# Autodesk Inventor assembly: GP5-200
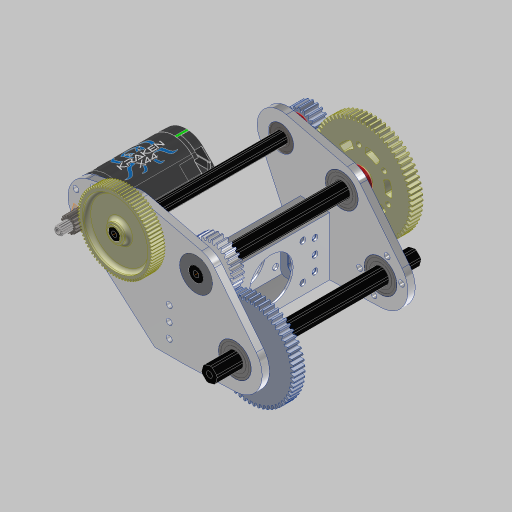
[picture p0: Inventor's stored thumbnail of the model, 512x512]
Saved by Autodesk Inventor 2023.5 (Build 275446000, 446)
## iProperties
Created: 2025-02-04
Part Number: GP5-200
Document SubType Name: Assembly
Designer: mavericks
Mass: 1428.35 g
Surface Area: 2144.98 cm^2
Volume: 477.65 cm^3
Density: 2.99036 g/cm^3
Author: mavericks
## Documents named in this file (21)
- C:\Users\slick\OneDrive\Desktop\2025-ReefScape---CAD\Gripper\GP5\GP5-200.iam
- C:\Users\slick\OneDrive\Desktop\2025-ReefScape---CAD\Gripper\GP5\GP5-001.ipt
- C:\Users\slick\OneDrive\Desktop\2025-ReefScape---CAD\Gripper\GP5\GP5-002.ipt
- C:\Users\slick\OneDrive\Desktop\2025-ReefScape---CAD\Gripper\GP5\GP5-004.ipt
- C:\Users\slick\OneDrive\Desktop\2025-ReefScape---CAD\COMMON PARTS\BEARINGS\13_75mm_1_2_ThunderHex_ID_x_1_125_OD_x_0_313_WD_Flanged_Bearing_217-4006_MIR.ipt
- C:\Users\slick\OneDrive\Desktop\2025-ReefScape---CAD\COMMON PARTS\MOTORS\WCP-0941 x44 Kracken.ipt
- C:\Users\slick\OneDrive\Desktop\2025-ReefScape---CAD\COMMON PARTS\GEARS\32 dp gear\WCP-1464.ipt
- C:\Users\slick\OneDrive\Desktop\2025-ReefScape---CAD\COMMON PARTS\GEARS\32 dp gear\80t_Aluminum_Spur_Gear_32_DP_3_8_Hex_Bore_217-5864.ipt
- C:\Users\slick\OneDrive\Desktop\2025-ReefScape---CAD\COMMON PARTS\GEARS\20dp .375 hex\20t_Aluminum_Spur_Gear_20_DP_3_8_Hex_Bore_217-2701.ipt
- C:\Users\slick\OneDrive\Desktop\2025-ReefScape---CAD\COMMON PARTS\GEARS\20dp .5 hex\66t_Aluminum_Spur_Gear_20_DP_1_2_Hex_Bore_VersaKeys_217-3223.ipt
- C:\Users\slick\OneDrive\Desktop\2025-ReefScape---CAD\COMMON PARTS\GEARS\20dp .5 hex\30t_Aluminum_Spur_Gear_20_DP_1_2_Hex_Bore_217-2705.ipt
- C:\Users\slick\OneDrive\Desktop\2025-ReefScape---CAD\COMMON PARTS\GEARS\20dp .5 hex\60t_Aluminum_Spur_Gear_20_DP_1_2_Hex_Bore_217-3574.ipt
- C:\Users\slick\OneDrive\Desktop\2025-ReefScape---CAD\Gripper\GP5\GP5-008.ipt
- C:\Users\slick\OneDrive\Desktop\2025-ReefScape---CAD\COMMON PARTS\BEARINGS\10_25mm_3_8_ThunderHex_ID_x_0_875_OD_x_0_280_WD_Flanged_Bearing_217-5829.ipt
- C:\Users\slick\OneDrive\Desktop\2025-ReefScape---CAD\Gripper\GP5\GP5-009.ipt
- C:\Users\slick\OneDrive\Desktop\2025-ReefScape---CAD\Gripper\GP5\GP5-010.ipt
- C:\Users\slick\OneDrive\Desktop\2025-ReefScape---CAD\Gripper\GP5\GP5-011.ipt
- C:\Users\slick\OneDrive\Desktop\2025-ReefScape---CAD\Gripper\GP5\GP5-020.ipt
- C:\Users\slick\OneDrive\Desktop\2025-ReefScape---CAD\Gripper\GP5\GP5-021.ipt
- C:\Users\slick\OneDrive\Desktop\2025-ReefScape---CAD\Gripper\GP5\GP5-022.ipt
- C:\Users\slick\OneDrive\Desktop\2025-ReefScape---CAD\COMMON PARTS\BEARINGS\0_500_ID_x_1_125_OD_x_0_313_WD_Flanged_Bearing_217-2731.ipt
## Components (26 placed, 20 different names)
1. GP5-001:1 — Flush:1, Flush:2, Flush:3, Flush:4, Flush:5, Mate:1
2. GP5-002:1 — Flush:2, Flush:3, Flush:4, Insert:3, Insert:4
3. GP5-002:2 — Flush:1, Flush:5, Mate:1, Insert:1, Insert:2
4. GP5-011:1 — Insert:3, Insert:4, Insert:5, Insert:6, Insert:13, Symmetry:1
5. GP5-004:2 — Insert:1, Insert:2, Insert:10, Mate:2, Mate:3, Insert:11, Insert:12, Insert:14, Symmetry:1
6. 0_500_ID_x_1_125_OD_x_0_313_WD_Flanged_Bearing_217-2731:1 — Insert:14, Flush:14, Mate:32, Mate:33
7. 13_75mm_1_2_ThunderHex_ID_x_1_125_OD_x_0_313_WD_Flanged_Bearing_217-4006_MIR:3 — Insert:10, Mate:12
8. 13_75mm_1_2_ThunderHex_ID_x_1_125_OD_x_0_313_WD_Flanged_Bearing_217-4006_MIR:5 — Insert:6, Mate:8, Mate:17, Mate:24
9. 13_75mm_1_2_ThunderHex_ID_x_1_125_OD_x_0_313_WD_Flanged_Bearing_217-4006_MIR:6 — Insert:5, Mate:18
10. WCP-0941 x44 Kracken:1 — Mate:2, Mate:3, Insert:11, Mate:4, Mate:5
11. WCP-1464:1 — Mate:4, Mate:5, Flush:6, Rotation:1
12. 80t_Aluminum_Spur_Gear_32_DP_3_8_Hex_Bore_217-5864:1 — Flush:6, Mate:13, Flush:9, Angle:1, Rotation:1
13. 20t_Aluminum_Spur_Gear_20_DP_3_8_Hex_Bore_217-2701:1 — Flush:7, Mate:14, Angle:2, Rotation:2, Flush:13
14. 66t_Aluminum_Spur_Gear_20_DP_1_2_Hex_Bore_VersaKeys_217-3223:1 — Mate:8, Flush:7, Angle:3, Rotation:2
15. 30t_Aluminum_Spur_Gear_20_DP_1_2_Hex_Bore_217-2705:1 — Flush:8, Angle:4, Rotation:3, Mate:30, Mate:33
16. 60t_Aluminum_Spur_Gear_20_DP_1_2_Hex_Bore_217-3574:1 — Flush:8, Mate:12, Angle:5, Rotation:3, Mate:29
17. GP5-008:1 — Mate:16, Flush:9, Angle:1, Angle:2, Mate:25, Mate:27, Flush:13
18. 10_25mm_3_8_ThunderHex_ID_x_0_875_OD_x_0_280_WD_Flanged_Bearing_217-5829:1 — Insert:12, Mate:13, Mate:16, Mate:26
19. 10_25mm_3_8_ThunderHex_ID_x_0_875_OD_x_0_280_WD_Flanged_Bearing_217-5829:2 — Insert:13, Mate:14, Mate:28
20. GP5-009:1 — Mate:17, Angle:3, Angle:4, Mate:20, Mate:23, Flush:14
21. GP5-010:1 — Mate:18, Angle:5, Mate:19, Mate:31
22. GP5-020:1 — Mate:19, Mate:29
23. GP5-020:2 — Mate:20, Mate:30, Mate:32
24. GP5-021:1 — Mate:23, Mate:24
25. GP5-022:1 — Mate:25, Mate:26
26. GP5-021:2 — Mate:27, Mate:28
## Relationships (56: Mate 25, Flush 11, Insert 11, Angle 5, RelateRotation 3, Symmetry 1)
- Flush:1: GP5-001:1 ↔ GP5-002:2
- Flush:2: GP5-001:1 ↔ GP5-002:1
- Flush:3: GP5-001:1 ↔ GP5-002:1
- Flush:4: GP5-001:1 ↔ GP5-002:1
- Flush:5: GP5-001:1 ↔ GP5-002:2
- Mate:1: GP5-001:1 ↔ GP5-002:2
- Insert:1: GP5-002:2 ↔ GP5-004:2
- Insert:2: GP5-002:2 ↔ GP5-004:2
- Insert:3: GP5-002:1 ↔ GP5-011:1
- Insert:4: GP5-002:1 ↔ GP5-011:1
- Insert:5: GP5-011:1 ↔ 13_75mm_1_2_ThunderHex_ID_x_1_125_OD_x_0_313_WD_Flanged_Bearing_217-4006_MIR:6
- Insert:6: GP5-011:1 ↔ 13_75mm_1_2_ThunderHex_ID_x_1_125_OD_x_0_313_WD_Flanged_Bearing_217-4006_MIR:5
- Insert:10: GP5-004:2 ↔ 13_75mm_1_2_ThunderHex_ID_x_1_125_OD_x_0_313_WD_Flanged_Bearing_217-4006_MIR:3
- Mate:2: GP5-004:2 ↔ WCP-0941 x44 Kracken:1
- Mate:3: GP5-004:2 ↔ WCP-0941 x44 Kracken:1
- Insert:11: GP5-004:2 ↔ WCP-0941 x44 Kracken:1
- Mate:4: WCP-0941 x44 Kracken:1 ↔ WCP-1464:1
- Mate:5 (3.175 mm): WCP-0941 x44 Kracken:1 ↔ WCP-1464:1
- Flush:6: WCP-1464:1 ↔ 80t_Aluminum_Spur_Gear_32_DP_3_8_Hex_Bore_217-5864:1
- Mate:8: 13_75mm_1_2_ThunderHex_ID_x_1_125_OD_x_0_313_WD_Flanged_Bearing_217-4006_MIR:5 ↔ 66t_Aluminum_Spur_Gear_20_DP_1_2_Hex_Bore_VersaKeys_217-3223:1
- Flush:7: 20t_Aluminum_Spur_Gear_20_DP_3_8_Hex_Bore_217-2701:1 ↔ 66t_Aluminum_Spur_Gear_20_DP_1_2_Hex_Bore_VersaKeys_217-3223:1
- Flush:8: 30t_Aluminum_Spur_Gear_20_DP_1_2_Hex_Bore_217-2705:1 ↔ 60t_Aluminum_Spur_Gear_20_DP_1_2_Hex_Bore_217-3574:1
- Mate:12: 13_75mm_1_2_ThunderHex_ID_x_1_125_OD_x_0_313_WD_Flanged_Bearing_217-4006_MIR:3 ↔ 60t_Aluminum_Spur_Gear_20_DP_1_2_Hex_Bore_217-3574:1
- Insert:12: GP5-004:2 ↔ 10_25mm_3_8_ThunderHex_ID_x_0_875_OD_x_0_280_WD_Flanged_Bearing_217-5829:1
- Insert:13: GP5-011:1 ↔ 10_25mm_3_8_ThunderHex_ID_x_0_875_OD_x_0_280_WD_Flanged_Bearing_217-5829:2
- Mate:13: 80t_Aluminum_Spur_Gear_32_DP_3_8_Hex_Bore_217-5864:1 ↔ 10_25mm_3_8_ThunderHex_ID_x_0_875_OD_x_0_280_WD_Flanged_Bearing_217-5829:1
- Mate:14: 20t_Aluminum_Spur_Gear_20_DP_3_8_Hex_Bore_217-2701:1 ↔ 10_25mm_3_8_ThunderHex_ID_x_0_875_OD_x_0_280_WD_Flanged_Bearing_217-5829:2
- Mate:16: GP5-008:1 ↔ 10_25mm_3_8_ThunderHex_ID_x_0_875_OD_x_0_280_WD_Flanged_Bearing_217-5829:1
- Flush:9: 80t_Aluminum_Spur_Gear_32_DP_3_8_Hex_Bore_217-5864:1 ↔ GP5-008:1
- Angle:1 (0 deg): 80t_Aluminum_Spur_Gear_32_DP_3_8_Hex_Bore_217-5864:1 ↔ GP5-008:1
- Angle:2 (0 deg): 20t_Aluminum_Spur_Gear_20_DP_3_8_Hex_Bore_217-2701:1 ↔ GP5-008:1
- Rotation:1 [RelateRotation] (5.3333 ul): WCP-1464:1 ↔ 80t_Aluminum_Spur_Gear_32_DP_3_8_Hex_Bore_217-5864:1
- Mate:17: 13_75mm_1_2_ThunderHex_ID_x_1_125_OD_x_0_313_WD_Flanged_Bearing_217-4006_MIR:5 ↔ GP5-009:1
- Mate:18: 13_75mm_1_2_ThunderHex_ID_x_1_125_OD_x_0_313_WD_Flanged_Bearing_217-4006_MIR:6 ↔ GP5-010:1
- Angle:3 (0 deg): 66t_Aluminum_Spur_Gear_20_DP_1_2_Hex_Bore_VersaKeys_217-3223:1 ↔ GP5-009:1
- Angle:4 (0 deg): 30t_Aluminum_Spur_Gear_20_DP_1_2_Hex_Bore_217-2705:1 ↔ GP5-009:1
- Angle:5 (0 deg): 60t_Aluminum_Spur_Gear_20_DP_1_2_Hex_Bore_217-3574:1 ↔ GP5-010:1
- Rotation:2 [RelateRotation] (3.3 ul): 20t_Aluminum_Spur_Gear_20_DP_3_8_Hex_Bore_217-2701:1 ↔ 66t_Aluminum_Spur_Gear_20_DP_1_2_Hex_Bore_VersaKeys_217-3223:1
- Rotation:3 [RelateRotation] (2 ul): 30t_Aluminum_Spur_Gear_20_DP_1_2_Hex_Bore_217-2705:1 ↔ 60t_Aluminum_Spur_Gear_20_DP_1_2_Hex_Bore_217-3574:1
- Mate:19: GP5-010:1 ↔ GP5-020:1
- Mate:20: GP5-009:1 ↔ GP5-020:2
- Mate:23: GP5-009:1 ↔ GP5-021:1
- Mate:24: 13_75mm_1_2_ThunderHex_ID_x_1_125_OD_x_0_313_WD_Flanged_Bearing_217-4006_MIR:5 ↔ GP5-021:1
- Mate:25: GP5-008:1 ↔ GP5-022:1
- Mate:26: 10_25mm_3_8_ThunderHex_ID_x_0_875_OD_x_0_280_WD_Flanged_Bearing_217-5829:1 ↔ GP5-022:1
- Mate:27: GP5-008:1 ↔ GP5-021:2
- Mate:28: 10_25mm_3_8_ThunderHex_ID_x_0_875_OD_x_0_280_WD_Flanged_Bearing_217-5829:2 ↔ GP5-021:2
- Mate:29: 60t_Aluminum_Spur_Gear_20_DP_1_2_Hex_Bore_217-3574:1 ↔ GP5-020:1
- Mate:30: 30t_Aluminum_Spur_Gear_20_DP_1_2_Hex_Bore_217-2705:1 ↔ GP5-020:2
- Flush:13: 20t_Aluminum_Spur_Gear_20_DP_3_8_Hex_Bore_217-2701:1 ↔ GP5-008:1
- Insert:14: GP5-004:2 ↔ 0_500_ID_x_1_125_OD_x_0_313_WD_Flanged_Bearing_217-2731:1
- Flush:14: 0_500_ID_x_1_125_OD_x_0_313_WD_Flanged_Bearing_217-2731:1 ↔ GP5-009:1
- Symmetry:1: GP5-011:1 ↔ GP5-004:2
- Mate:31: GP5-010:1
- Mate:32: 0_500_ID_x_1_125_OD_x_0_313_WD_Flanged_Bearing_217-2731:1 ↔ GP5-020:2
- Mate:33: 0_500_ID_x_1_125_OD_x_0_313_WD_Flanged_Bearing_217-2731:1 ↔ 30t_Aluminum_Spur_Gear_20_DP_1_2_Hex_Bore_217-2705:1
